# Autodesk Inventor assembly: CartWhole
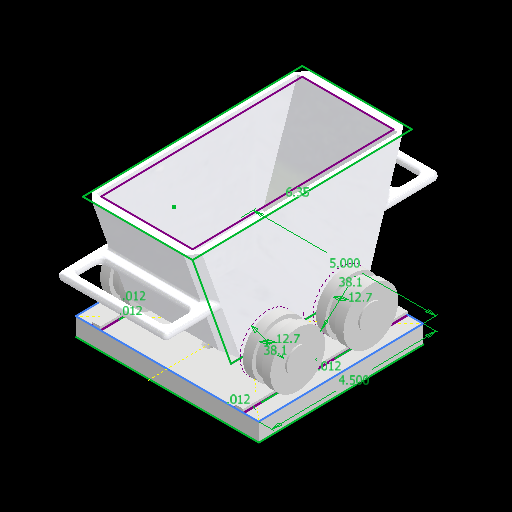
[picture p0: Inventor's stored thumbnail of the model, 512x512]
Saved by Autodesk Inventor 2025 (Build 290162000, 162)
## iProperties
Created: 2025-03-04
Part Number: CartWhole
Document SubType Name: Assembly
Designer: Trevor
Author: Trevor
## Documents named in this file (6)
- C:\Users\Trevor\Documents\GitHub\USA-Robotic-Club-2024\CartWhole.iam
- C:\Users\Trevor\Documents\GitHub\USA-Robotic-Club-2024\CartMK1.ipt
- C:\Users\Trevor\Documents\GitHub\USA-Robotic-Club-2024\Cart Wheel.ipt
- C:\Users\Trevor\Documents\GitHub\USA-Robotic-Club-2024\CartWheelCap.ipt
- C:\Users\Trevor\Documents\GitHub\USA-Robotic-Club-2024\Track Piece.ipt
- C:\Users\Trevor\Documents\GitHub\USA-Robotic-Club-2024\CartTrack.ipt
## Components (11 placed, 5 different names)
1. CartMK1:1 — Mate:1, Mate:2, Mate:3, Mate:4, Flush:1, Flush:2, Flush:3, Flush:4, Flush:5, Mate:5, Mate:6, Mate:7, Mate:8, Mate:9, Angle:1, Flush:7
2. Cart Wheel:1 — Mate:1, Flush:2
3. Cart Wheel:2 — Mate:2, Flush:1
4. Cart Wheel:3 — Mate:4, Flush:4, Tangent:1
5. Cart Wheel:4 — Mate:3, Flush:3
6. CartWheelCap:1 — Flush:5
7. CartWheelCap:2 — Mate:6, Mate:8
8. CartWheelCap:3 — Mate:5
9. CartWheelCap:4 — Mate:7, Mate:9
10. Track Piece:1 — Flush:6
11. CartTrack:1 — Flush:8
## Relationships (19: Mate 9, Flush 8, Angle 1, Tangent 1)
- Mate:1: CartMK1:1 ↔ Cart Wheel:1
- Mate:2: CartMK1:1 ↔ Cart Wheel:2
- Mate:3: CartMK1:1 ↔ Cart Wheel:4
- Mate:4: CartMK1:1 ↔ Cart Wheel:3
- Flush:1: CartMK1:1 ↔ Cart Wheel:2
- Flush:2: CartMK1:1 ↔ Cart Wheel:1
- Flush:3: CartMK1:1 ↔ Cart Wheel:4
- Flush:4: CartMK1:1 ↔ Cart Wheel:3
- Flush:5: CartMK1:1 ↔ CartWheelCap:1
- Mate:5: CartMK1:1 ↔ CartWheelCap:3
- Mate:6: CartMK1:1 ↔ CartWheelCap:2
- Mate:7: CartMK1:1 ↔ CartWheelCap:4
- Mate:8: CartMK1:1 ↔ CartWheelCap:2
- Mate:9: CartMK1:1 ↔ CartWheelCap:4
- Angle:1 (0 deg): CartMK1:1
- Tangent:1: Cart Wheel:3
- Flush:6: Track Piece:1
- Flush:7: CartMK1:1
- Flush:8: CartTrack:1
